# Autodesk Inventor assembly: AX-12
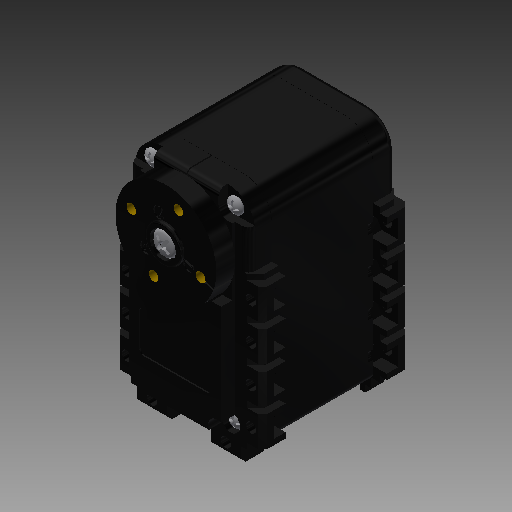
[picture p0: Inventor's stored thumbnail of the model, 512x512]
Saved by Autodesk Inventor 2019 (Build 230136000, 136)
## iProperties
Created: 2011-05-31
Part Number: AX-12
Material: Типовые
Document SubType Name: Assembly
Designer: Петров Иван
Mass: 45.9038 g
Surface Area: 138.627 cm^2
Volume: 43.3506 cm^3
Density: 1.0589 g/cm^3
Sending System: PRO/ENGINEER BY PARAMETRIC TECHNOLOGY CORPORATION, 2009060
Preprocessor: PRO/ENGINEER BY PARAMETRIC TECHNOLOGY CORPORATION, 2009060
Title: AX12_ASM
Author: yun
Revision Number: 3LAST_VERSION
## Documents named in this file (7)
- E:\IVAN\Kvantoriada2019\optimal_gripper\hardware\Стандартные изделия\Сервомотор Dynamixel AX-12A\AX-12.iam
- E:\IVAN\Kvantoriada2019\optimal_gripper\hardware\Стандартные изделия\Сервомотор Dynamixel AX-12A\ASSY_DUMMY__.ipt
- E:\IVAN\Kvantoriada2019\optimal_gripper\hardware\Стандартные изделия\Сервомотор Dynamixel AX-12A\ASSY_GEAR-WHEEL__.ipt
- E:\IVAN\Kvantoriada2019\optimal_gripper\hardware\Стандартные изделия\Сервомотор Dynamixel AX-12A\DX124_SCREW-COVER__.ipt
- E:\IVAN\Kvantoriada2019\optimal_gripper\hardware\Стандартные изделия\Сервомотор Dynamixel AX-12A\099990987___.ipt
- E:\IVAN\Kvantoriada2019\optimal_gripper\hardware\Стандартные изделия\Сервомотор Dynamixel AX-12A\DX124_HORN1__.ipt
- E:\IVAN\Kvantoriada2019\optimal_gripper\hardware\Стандартные изделия\Сервомотор Dynamixel AX-12A\PHS_M3X10__.ipt
## Components (10 placed, 10 different names)
1. ASSY_DUMMY___0 — Совмещение:1, Вставка:1, Совмещение:2, Вставка:2, Совмещение:3, Вставка:3, Совмещение:4, Вставка:4, Совмещение:5, Совмещение:6
2. ASSY_GEAR-WHEEL___1 — Совмещение:5, Совмещение:6, Совмещение:8, Совмещение:9, Направление навивки:1
3. DX124_SCREW-COVER___2 — Совмещение:1, Вставка:1
4. DX124_SCREW-COVER___3 — Совмещение:2, Вставка:2
5. DX124_SCREW-COVER___4 — Совмещение:3, Вставка:3
6. DX124_SCREW-COVER___5 — Совмещение:4, Вставка:4
7. 099990987____6
8. 099990987____7
9. DX124_HORN1___8 — Совмещение:8, Совмещение:9, Направление навивки:1, Совмещение:10, Совмещение:11
10. PHS_M3X10___9 — Совмещение:10, Совмещение:11
## Relationships (15: Mate 10, Insert 4, RelateRotation 1)
- Совмещение:1 [Mate]: ASSY_DUMMY___0 ↔ DX124_SCREW-COVER___2
- Вставка:1 [Insert]: ASSY_DUMMY___0 ↔ DX124_SCREW-COVER___2
- Совмещение:2 [Mate]: ASSY_DUMMY___0 ↔ DX124_SCREW-COVER___3
- Вставка:2 [Insert]: ASSY_DUMMY___0 ↔ DX124_SCREW-COVER___3
- Совмещение:3 [Mate]: ASSY_DUMMY___0 ↔ DX124_SCREW-COVER___4
- Вставка:3 [Insert]: ASSY_DUMMY___0 ↔ DX124_SCREW-COVER___4
- Совмещение:4 [Mate]: ASSY_DUMMY___0 ↔ DX124_SCREW-COVER___5
- Вставка:4 [Insert]: ASSY_DUMMY___0 ↔ DX124_SCREW-COVER___5
- Совмещение:5 [Mate]: ASSY_DUMMY___0 ↔ ASSY_GEAR-WHEEL___1
- Совмещение:6 [Mate]: ASSY_DUMMY___0 ↔ ASSY_GEAR-WHEEL___1
- Совмещение:8 [Mate]: ASSY_GEAR-WHEEL___1 ↔ DX124_HORN1___8
- Совмещение:9 [Mate]: ASSY_GEAR-WHEEL___1 ↔ DX124_HORN1___8
- Направление навивки:1 [RelateRotation] (1 ul): ASSY_GEAR-WHEEL___1 ↔ DX124_HORN1___8
- Совмещение:10 [Mate]: DX124_HORN1___8 ↔ PHS_M3X10___9
- Совмещение:11 [Mate]: DX124_HORN1___8 ↔ PHS_M3X10___9
